# Autodesk Inventor assembly: WheelAssembly
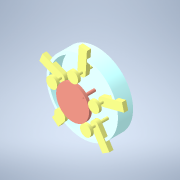
[picture p0: Inventor's stored thumbnail of the model, 180x180]
Saved by Autodesk Inventor 2020.1 (Build 241239000, 239)
## iProperties
Created: 2019-11-14
Part Number: WheelAssembly
Document SubType Name: Assembly
Designer: Ali
Author: Ali
## Documents named in this file (5)
- F:\Inventor_Projects\ARCS\WheelAssembly.iam
- F:\Inventor_Projects\ARCS\Wheel.ipt
- F:\Inventor_Projects\ARCS\mainGear.ipt
- F:\Inventor_Projects\ARCS\smallGear.ipt
- F:\Inventor_Projects\ARCS\Excel\Parameters.xlsx
## Components (7 placed, 3 different names)
1. Wheel:1 — Flush:2, Insert:2, Insert:3
2. mainGear:1 — Insert:3, Rotation:1
3. smallGear:1 — Flush:2, Insert:2, Rotation:1
4. smallGear:2
5. smallGear:3
6. smallGear:4
7. smallGear:5
## Component patterns: (5 elements, first: smallGear:1)
## Relationships (4: Insert 2, Flush 1, RelateRotation 1)
- Flush:2: Wheel:1 ↔ smallGear:1
- Insert:2: Wheel:1 ↔ smallGear:1
- Insert:3 (-25.4 mm): Wheel:1 ↔ mainGear:1
- Rotation:1 [RelateRotation] (0.3333 ul): mainGear:1 ↔ smallGear:1
## Named parameters: wheelR = 76.2 mm, wheelDepth = 50.8 mm, wheelThickness = 6.35 mm, farFromCenter = 50.8 mm, mainHole = 6.858 mm, smallHoles = 6.858 mm, gearShaft = 6.35 mm, mainGear = 38.1 mm, smallGear = 12.7 mm, numberOfSmallGears = 5, smallGearLength = 50.8 mm, mainGearLength = 76.2 mm, gearThickness = 6.35 mm, swivelLegExtentions = 19.05 mm, swivelBaseDiameter = 19.05 mm, swivelLegLength = 49.13565 mm, swivelLegThickness = 19.05 mm, gearR = 3, gearRatio = 3
